# Autodesk Inventor assembly: base frame
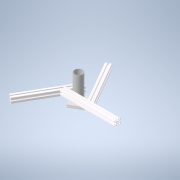
[picture p0: Inventor's stored thumbnail of the model, 180x180]
Saved by Autodesk Inventor 2021 (Build 250183000, 183)
## iProperties
Created: 2022-09-08
Part Number: base frame
Document SubType Name: Assembly
Designer: Administrator
Title: base frame
Author: Administrator
## Documents named in this file (9)
- C:\Git\PhD\Inventor\GTPR_toBeBuilt\base frame.iam
- C:\Git\PhD\Inventor\GTPR_toBeBuilt\125mm od pvc pipe v1.ipt
- C:\Git\PhD\Inventor\GTPR_toBeBuilt\upperClamp.ipt
- C:\Git\PhD\Inventor\GTPR_toBeBuilt\item_7000009_Profile_8_40x40_E_L=400.ipt
- C:\Git\PhD\Inventor\GTPR_toBeBuilt\heco_FL-060-006-4 v1.ipt
- C:\Git\PhD\Inventor\GTPR_toBeBuilt\motor mount lower.ipt
- C:\Git\PhD\Inventor\GTPR_toBeBuilt\NEMA_34_12Nm v1.ipt
- C:\Git\PhD\Inventor\GTPR_toBeBuilt\motor mount middle.ipt
- C:\Git\PhD\Inventor\GTPR_toBeBuilt\motor mount upper.ipt
## Components (14 placed, 8 different names)
1. 125mm od pvc pipe v1:1 — Mate:1, Mate:2, Mate:3, Flush:1, Mate:12, Mate:13
2. upperClamp:1 — Mate:1
3. upperClamp:2 — Mate:2
4. upperClamp:3 — Mate:3, Flush:1
5. item_7000009_Profile_8_40x40_E_L=400:1 — Mate:10, Mate:30, Flush:8, Mate:31
6. item_7000009_Profile_8_40x40_E_L=400:2 — Mate:10, Mate:11, Mate:33, Flush:9, Mate:34
7. item_7000009_Profile_8_40x40_E_L=400:3 — Mate:11, Angle:3, Mate:28, Flush:7, Mate:29
8. heco_FL-060-006-4 v1:1 — Mate:12, Mate:13
9. motor mount lower:1 — Mate:16, Mate:19, Mate:30, Flush:8, Mate:31, Mate:32
10. NEMA_34_12Nm v1:1 — Mate:16, Mate:19, Mate:32
11. motor mount middle:1 — Mate:24, Mate:25, Mate:33, Flush:9, Mate:34
12. motor mount upper:1 — Mate:26, Mate:27, Mate:28, Flush:7, Mate:29
13. NEMA_34_12Nm v1:2 — Mate:26, Mate:27
14. NEMA_34_12Nm v1:3 — Mate:24, Mate:25
## Relationships (36: Mate 26, Flush 7, Angle 3)
- Mate:1: 125mm od pvc pipe v1:1 ↔ upperClamp:1
- Mate:2: 125mm od pvc pipe v1:1 ↔ upperClamp:2
- Mate:3: 125mm od pvc pipe v1:1 ↔ upperClamp:3
- Flush:1: 125mm od pvc pipe v1:1 ↔ upperClamp:3
- [Mate]: upperClamp:3 ↔ item_7000009_Profile_8_40x40_E_L=400:1
- [Mate]: upperClamp:3 ↔ item_7000009_Profile_8_40x40_E_L=400:1
- [Flush]: upperClamp:3 ↔ item_7000009_Profile_8_40x40_E_L=400:1
- [Mate]: upperClamp:1 ↔ item_7000009_Profile_8_40x40_E_L=400:2
- [Flush]: upperClamp:1 ↔ item_7000009_Profile_8_40x40_E_L=400:2
- [Mate]: upperClamp:1 ↔ item_7000009_Profile_8_40x40_E_L=400:2
- [Mate]: upperClamp:2 ↔ item_7000009_Profile_8_40x40_E_L=400:3
- [Flush]: upperClamp:2 ↔ item_7000009_Profile_8_40x40_E_L=400:3
- [Mate]: upperClamp:2 ↔ item_7000009_Profile_8_40x40_E_L=400:3
- [Angle] (120 deg): item_7000009_Profile_8_40x40_E_L=400:1 ↔ item_7000009_Profile_8_40x40_E_L=400:2
- [Angle] (-120 deg): item_7000009_Profile_8_40x40_E_L=400:2 ↔ item_7000009_Profile_8_40x40_E_L=400:3
- Mate:10: item_7000009_Profile_8_40x40_E_L=400:1 ↔ item_7000009_Profile_8_40x40_E_L=400:2
- Mate:11: item_7000009_Profile_8_40x40_E_L=400:2 ↔ item_7000009_Profile_8_40x40_E_L=400:3
- Mate:12: 125mm od pvc pipe v1:1 ↔ heco_FL-060-006-4 v1:1
- Mate:13: 125mm od pvc pipe v1:1 ↔ heco_FL-060-006-4 v1:1
- Angle:3 (0 deg): item_7000009_Profile_8_40x40_E_L=400:3
- Mate:16: motor mount lower:1 ↔ NEMA_34_12Nm v1:1
- Mate:19: motor mount lower:1 ↔ NEMA_34_12Nm v1:1
- Mate:24: motor mount middle:1 ↔ NEMA_34_12Nm v1:3
- Mate:25: motor mount middle:1 ↔ NEMA_34_12Nm v1:3
- Mate:26: motor mount upper:1 ↔ NEMA_34_12Nm v1:2
- Mate:27: motor mount upper:1 ↔ NEMA_34_12Nm v1:2
- Mate:28: item_7000009_Profile_8_40x40_E_L=400:3 ↔ motor mount upper:1
- Flush:7: item_7000009_Profile_8_40x40_E_L=400:3 ↔ motor mount upper:1
- Mate:29: item_7000009_Profile_8_40x40_E_L=400:3 ↔ motor mount upper:1
- Mate:30: item_7000009_Profile_8_40x40_E_L=400:1 ↔ motor mount lower:1
- Flush:8: item_7000009_Profile_8_40x40_E_L=400:1 ↔ motor mount lower:1
- Mate:31: item_7000009_Profile_8_40x40_E_L=400:1 ↔ motor mount lower:1
- Mate:32: motor mount lower:1 ↔ NEMA_34_12Nm v1:1
- Mate:33: item_7000009_Profile_8_40x40_E_L=400:2 ↔ motor mount middle:1
- Flush:9: item_7000009_Profile_8_40x40_E_L=400:2 ↔ motor mount middle:1
- Mate:34: item_7000009_Profile_8_40x40_E_L=400:2 ↔ motor mount middle:1
